# Autodesk Inventor assembly: LS2_LEDs
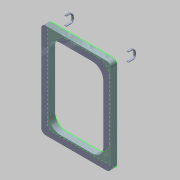
[picture p0: Inventor's stored thumbnail of the model, 180x180]
Saved by Autodesk Inventor 2019.3 (Build 233278000, 278)
## iProperties
Created: 2019-04-11
Part Number: LS2_LEDs
Document SubType Name: Assembly
Designer: Varga Daniel
Author: Varga Daniel
## Documents named in this file (5)
- C:\!_Dani\!_cloud\OneDrive\!_munka\Revolution\RevvyDemoKit\Structural parts\Demonstrations\Kickstarter videos\Brain pcb\minorParts\LS2_LEDs.iam
- C:\!_Dani\!_cloud\OneDrive\!_munka\Revolution\RevvyDemoKit\Structural parts\Demonstrations\Kickstarter videos\Brain pcb\minorParts\AS01508AO-SC-R.ipt
- C:\!_Dani\!_cloud\OneDrive\!_munka\Revolution\RevvyDemoKit\Structural parts\Demonstrations\Kickstarter videos\Brain pcb\minorParts\AS01508AO-SC-R_1.ipt
- C:\!_Dani\!_cloud\OneDrive\!_munka\Revolution\RevvyDemoKit\Structural parts\Demonstrations\Kickstarter videos\Brain pcb\minorParts\AS01508AO-SC-R_2.ipt
- C:\!_Dani\!_cloud\OneDrive\!_munka\Revolution\RevvyDemoKit\Structural parts\Demonstrations\Kickstarter videos\Brain pcb\publish\LS2_LEDs_patch.ipt
## Components (4 placed, 4 different names)
1. AS01508AO-SC-R
2. AS01508AO-SC-R_1 — Flush:1, Flush:2
3. AS01508AO-SC-R_2
4. LS2_LEDs_patch:1 — Flush:1, Flush:2
## Relationships (2: Flush 2)
- Flush:1: AS01508AO-SC-R_1 ↔ LS2_LEDs_patch:1
- Flush:2: AS01508AO-SC-R_1 ↔ LS2_LEDs_patch:1
